# Autodesk Inventor assembly: Pedal_tube
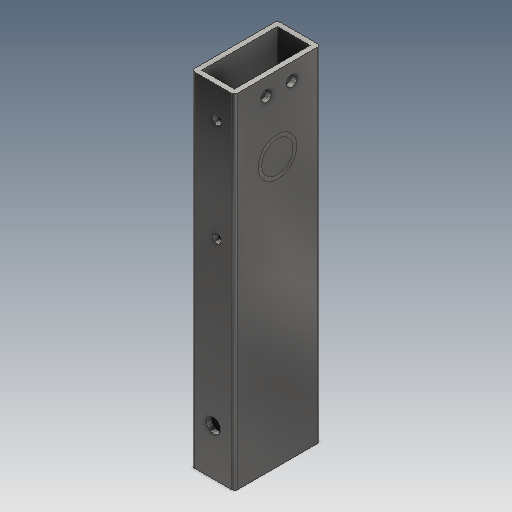
[picture p0: Inventor's stored thumbnail of the model, 512x512]
Saved by Autodesk Inventor 2020 (Build 240168000, 168)
## iProperties
Created: 2019-05-19
Part Number: Pedal_tube
Document SubType Name: Weldment
Designer: chitl
Weld Material: Steel, Mild, Welded
Mass: 291.407 g
Surface Area: 342.642 cm^2
Volume: 37.122 cm^3
Density: 7.85 g/cm^3
Author: chitl
## Documents named in this file (3)
- C:\Users\chitl\Desktop\OneWheel\Wheel Assembled\Pedal\Vertical Tube\Pedal_tube.iam
- C:\Users\chitl\Desktop\OneWheel\Wheel Assembled\Pedal\Vertical Tube\Pedal_Steel_1.5_0.75.ipt
- C:\Users\chitl\Desktop\OneWheel\Wheel Assembled\Pedal\Vertical Tube\Sleeve_0.5.ipt
## Components (2 placed, 2 different names)
1. Pedal_Steel_1.5_0.75:1 — Rigid:1
2. Sleeve_0.5:1 — Rigid:1
## Relationships (1: WeldJoint 1)
- Rigid:1 [WeldJoint]: Pedal_Steel_1.5_0.75:1 ↔ Sleeve_0.5:1
